# Autodesk Inventor assembly: Battery
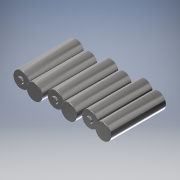
[picture p0: Inventor's stored thumbnail of the model, 180x180]
Saved by Autodesk Inventor 2018 (Build 220112000, 112)
## iProperties
Created: 2017-12-26
Part Number: Battery
Material: 一般
Description: STEP AP214
Document SubType Name: Assembly
Designer: ku_sk
Mass: 144 g
Surface Area: 146.842 cm^2
Volume: 44.9932 cm^3
Density: 3.20049 g/cm^3
Sending System: SolidWorks 2016
Preprocessor: SwSTEP 2.0
Title: balboa-balancing-robot-kit.step
Revision Number: ANY
## Documents named in this file (2)
- D:\Inventor\Balboa32U4-CAD\parts\Battery\Battery.iam
- D:\Inventor\Balboa32U4-CAD\parts\Battery\parts\AA_Battery.ipt
## Components (6 placed, 1 different names)
1. AA_Battery:1
2. AA_Battery:3
3. AA_Battery:4
4. AA_Battery:2
5. AA_Battery:5
6. AA_Battery:6
## Component patterns: (3 elements, first: AA_Battery:1), (3 elements, first: AA_Battery:2)
